# Autodesk Inventor assembly: Rotrkopf
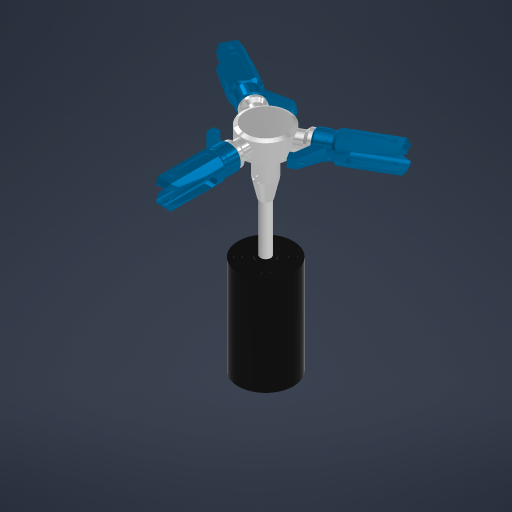
[picture p0: Inventor's stored thumbnail of the model, 512x512]
Saved by Autodesk Inventor 2023.2 (Build 272271000, 271)
## iProperties
Created: 2023-03-31
Part Number: Rotrkopf
Document SubType Name: Assembly
Designer: tadeu
Author: tadeu
## Documents named in this file (5)
- C:\Users\tadeu\Documents\0 Nerdy\CAD\Inventor\Studium\5. Semester\NWPL\WKA\Bauteile\Rotorkopf\Rotrkopf.iam
- C:\Users\tadeu\Documents\0 Nerdy\CAD\Inventor\Studium\5. Semester\NWPL\WKA\Bauteile\Rotorkopf\RotorKopf_Hub.ipt
- C:\Users\tadeu\Documents\0 Nerdy\CAD\Inventor\Studium\5. Semester\NWPL\WKA\Bauteile\Rotorkopf\RotorArm.ipt
- C:\Users\tadeu\Documents\0 Nerdy\CAD\Inventor\Studium\5. Semester\NWPL\WKA\Bauteile\Rotorkopf\Welle.ipt
- C:\Users\tadeu\Documents\0 Nerdy\CAD\Inventor\Studium\5. Semester\NWPL\WKA\Bauteile\Technik\Generator\Generator.ipt
## Components (6 placed, 4 different names)
1. Welle:1 — Drehbar:1, Starr:1
2. RotorKopf_Hub:1 — Drehbar:1, Drehbar:2
3. Generator:1 — Starr:1
4. RotorArm:1 — Drehbar:2
5. RotorArm:2
6. RotorArm:3
## Component patterns: (3 elements, first: RotorArm:1)
## Relationships (3: RevoluteJoint 2, WeldJoint 1)
- Drehbar:1 [RevoluteJoint]: Welle:1 ↔ RotorKopf_Hub:1
- Drehbar:2 [RevoluteJoint]: RotorKopf_Hub:1 ↔ RotorArm:1
- Starr:1 [WeldJoint]: Welle:1 ↔ Generator:1
